# Autodesk Inventor assembly: Sub system 3 assembly
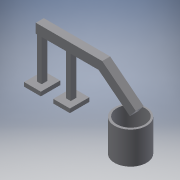
[picture p0: Inventor's stored thumbnail of the model, 180x180]
Saved by Autodesk Inventor 2019 (Build 230136000, 136)
## iProperties
Created: 2020-04-19
Part Number: Sub system 3 assembly
Document SubType Name: Assembly
Designer: Adityan Matthew
Author: Adityan Matthew
## Documents named in this file (3)
- D:\Sub system 3 assembly.iam
- D:\int.ipt
- D:\int 3.ipt
## Components (3 placed, 2 different names)
1. int:1 — Rigid:1, Rigid:2
2. int 3:1 — Rigid:2
3. int 3:2 — Rigid:1
## Relationships (2: WeldJoint 2)
- Rigid:1 [WeldJoint]: int:1 ↔ int 3:2
- Rigid:2 [WeldJoint]: int:1 ↔ int 3:1
